# Autodesk Inventor assembly: Curved Assembly
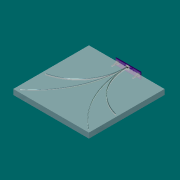
[picture p0: Inventor's stored thumbnail of the model, 180x180]
Saved by Autodesk Inventor 2016 (Build 200138000, 138)
## iProperties
Created: 2015-08-14
Part Number: Curved Assembly
Document SubType Name: Assembly
Designer: Cosmic
Author: Cosmic
## Documents named in this file (8)
- C:\Users\Cosmic\Documents\Inventor\SiPm ScintillatorTest Kit\Curved Assembly.iam
- C:\Users\Cosmic\Documents\Inventor\SiPm ScintillatorTest Kit\Scintillator Tile Tree.ipt
- C:\Users\Cosmic\Documents\Inventor\SiPm ScintillatorTest Kit\Four Fiber Bundle.iam
- C:\Users\Cosmic\Documents\Inventor\MPPC Sensor Board\MPPC Sensor V4 Populated.iam
- C:\Users\Cosmic\Documents\Inventor\Content Center Files\R2016\en-US\ANSI B18.6.7M(00)\ANSI B18.6.7M - M3x0.5 x 8(4).ipt
- C:\Users\Cosmic\Documents\Inventor\SiPm ScintillatorTest Kit\2mm spacer 93657A201.ipt
- C:\Users\Cosmic\Documents\Inventor\SiPm ScintillatorTest Kit\M3 Washer 95225A315.ipt
- C:\Users\Cosmic\Documents\Inventor\SiPm ScintillatorTest Kit\Scintillator.xlsx
## Components (9 placed, 6 different names)
1. Scintillator Tile Tree:1 — Angle:1, Tangent:1, Tangent:2, Flush:1, Mate:14, Mate:17, Mate:18
2. Four Fiber Bundle:1 [sub-assembly] — Angle:1, Tangent:1, Tangent:2, Flush:1
3. MPPC Sensor V4 Populated:1 [sub-assembly] — Mate:1, Mate:2, Mate:3, Mate:4, Mate:12, Mate:15
4. Cross Recessed Pan Head Machine Screw - Type I - Metric M3x0.5 x 8:1 — Mate:2, Mate:4, Mate:8, Mate:10, Mate:18
5. Cross Recessed Pan Head Machine Screw - Type I - Metric M3x0.5 x 8:2 — Mate:1, Mate:3, Mate:9, Mate:11, Mate:17
6. 2mm spacer 93657A201:1 — Mate:8, Mate:16
7. 2mm spacer 93657A201:2 — Mate:9, Mate:13, Mate:14
8. M3 Washer 95225A315:1 — Mate:10, Mate:15, Mate:16
9. M3 Washer 95225A315:2 — Mate:11, Mate:12, Mate:13
## Relationships (19: Mate 15, Tangent 2, Angle 1, Flush 1)
- Angle:1 (-90 deg): Scintillator Tile Tree:1 ↔ Four Fiber Bundle:1
- Tangent:1 (0.15 mm): Scintillator Tile Tree:1 ↔ Four Fiber Bundle:1
- Tangent:2 (0.15 mm): Scintillator Tile Tree:1 ↔ Four Fiber Bundle:1
- Flush:1: Scintillator Tile Tree:1 ↔ Four Fiber Bundle:1
- Mate:1: MPPC Sensor V4 Populated:1 ↔ Cross Recessed Pan Head Machine Screw - Type I - Metric M3x0.5 x 8:2
- Mate:2: MPPC Sensor V4 Populated:1 ↔ Cross Recessed Pan Head Machine Screw - Type I - Metric M3x0.5 x 8:1
- Mate:3: MPPC Sensor V4 Populated:1 ↔ Cross Recessed Pan Head Machine Screw - Type I - Metric M3x0.5 x 8:2
- Mate:4: MPPC Sensor V4 Populated:1 ↔ Cross Recessed Pan Head Machine Screw - Type I - Metric M3x0.5 x 8:1
- Mate:8: Cross Recessed Pan Head Machine Screw - Type I - Metric M3x0.5 x 8:1 ↔ 2mm spacer 93657A201:1
- Mate:9: Cross Recessed Pan Head Machine Screw - Type I - Metric M3x0.5 x 8:2 ↔ 2mm spacer 93657A201:2
- Mate:10: Cross Recessed Pan Head Machine Screw - Type I - Metric M3x0.5 x 8:1 ↔ M3 Washer 95225A315:1
- Mate:11: Cross Recessed Pan Head Machine Screw - Type I - Metric M3x0.5 x 8:2 ↔ M3 Washer 95225A315:2
- Mate:12: MPPC Sensor V4 Populated:1 ↔ M3 Washer 95225A315:2
- Mate:13: 2mm spacer 93657A201:2 ↔ M3 Washer 95225A315:2
- Mate:14: Scintillator Tile Tree:1 ↔ 2mm spacer 93657A201:2
- Mate:15: MPPC Sensor V4 Populated:1 ↔ M3 Washer 95225A315:1
- Mate:16: 2mm spacer 93657A201:1 ↔ M3 Washer 95225A315:1
- Mate:17: Scintillator Tile Tree:1 ↔ Cross Recessed Pan Head Machine Screw - Type I - Metric M3x0.5 x 8:2
- Mate:18: Scintillator Tile Tree:1 ↔ Cross Recessed Pan Head Machine Screw - Type I - Metric M3x0.5 x 8:1
## Named parameters: OpticalFiberClearence = 0.15 mm, MPPCClearence = 0.075 mm, FiberSensorClerence = 0.5 mm, OpticalFiberDiameter = 1 mm, ScintillatorThickness = 10 mm, SmallTrackDiameter = 175 mm, LargeTrackRatio = 3, ScintillatorEdgeClearence = 3 mm, ScintillatorWidth = 145 mm, ScintillatorHeight = 145 mm, ShallowTrackDepth = 1.3 mm, MPPCSensorClearence = 1.45 mm, MPPCSensorOffsett = 2.105 mm, MPPCWidth = 5.9 mm, MPPCHeight = 6.55 mm, FiberEdgeOffsett = 5 mm, MPPCDepth = 0 mm, LongFiberAngle = 30 deg, ShortFiberAngle = 78 deg, LoopLargeTrackRatio = 1.1, LoopSmallTrackDiameter = 90 mm, MountingScrewOffsett = 20 mm, MountingScrewDepth = 4 mm
